# Autodesk Inventor assembly: wing_MIR
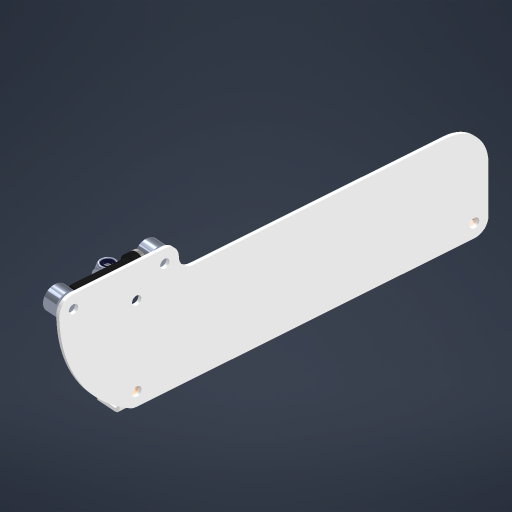
[picture p0: Inventor's stored thumbnail of the model, 512x512]
Saved by Autodesk Inventor 2024 (Build 280153000, 153)
## iProperties
Created: 2023-11-03
Part Number: wing_MIR
Document SubType Name: Assembly
Designer: avere
Author: avere
## Documents named in this file (11)
- C:\Users\avere\Documents\rbp_cad\zoomba_v0.1\chassis\wing_MIR.iam
- C:\Users\avere\Documents\rbp_cad\zoomba_v0.1\chassis\custom_parts\sled_MIR.ipt
- C:\Users\avere\Documents\rbp_cad\VEX-CAD-Inventor-1.41\Motion\Shaft LS\Shaft Collar ipts\Shaft Collar No Screw_MIR.ipt
- C:\Users\avere\Documents\rbp_cad\VEX-CAD-Inventor-1.41\Structure\Angle\Aluminum 1x1\Alu Angle 1x1x13_MIR.ipt
- C:\Users\avere\Documents\rbp_cad\VEX-CAD-Inventor-1.41\Structure\Standoff\Standoff 1.00.ipt
- C:\Users\avere\Documents\rbp_cad\VEX-CAD-Inventor-1.41\Structure\Standoff.ipt
- C:\Users\avere\Documents\rbp_cad\VEX-CAD-Inventor-1.41\Motion\Spacers\Spacer Nylon .375 OD\NSpacer .375 OD x .125.ipt
- C:\Users\avere\Documents\rbp_cad\VEX-CAD-Inventor-1.41\Motion\Spacers\Spacer Nylon .375 OD.ipt
- C:\Users\avere\Documents\rbp_cad\VEX-CAD-Inventor-1.41\Motion\Spacers\Washer Steel\SWasher .375 OD x .062500.ipt
- C:\Users\avere\Documents\rbp_cad\VEX-CAD-Inventor-1.41\Motion\Spacers\Washer Steel.ipt
- C:\Users\avere\Documents\rbp_cad\VEX-CAD-Inventor-1.41\Structure\Hardware\Nut Thin Nylock_MIR.ipt
## Components (10 placed, 7 different names)
1. sled_MIR:1 — Insert:10, Mate:4, Insert:11, Mate:5
2. Shaft Collar No Screw_MIR:1 — Insert:9, Insert:12
3. Shaft Collar No Screw_MIR:2 — Insert:9, Insert:8
4. Alu Angle 1x1x13_MIR:1 — Insert:10, Mate:4, Insert:12
5. Shaft Collar No Screw_MIR:3 — Mate:3, Insert:5, Insert:11
6. Shaft Collar No Screw_MIR:4 — Mate:3, Mate:5
7. Standoff 1.00:1 — Insert:5, Insert:4
8. NSpacer .375 OD x .125:1 — Insert:4, Insert:3
9. SWasher .375 OD x .062500:1 — Insert:3
10. Nut Thin Nylock_MIR:1 — Insert:8
## Relationships (11: Insert 8, Mate 3)
- Insert:9 (31.75 mm): Shaft Collar No Screw_MIR:1 ↔ Shaft Collar No Screw_MIR:2
- Mate:3: Shaft Collar No Screw_MIR:3 ↔ Shaft Collar No Screw_MIR:4
- Insert:5: Shaft Collar No Screw_MIR:3 ↔ Standoff 1.00:1
- Insert:4: Standoff 1.00:1 ↔ NSpacer .375 OD x .125:1
- Insert:3: NSpacer .375 OD x .125:1 ↔ SWasher .375 OD x .062500:1
- Insert:8: Shaft Collar No Screw_MIR:2 ↔ Nut Thin Nylock_MIR:1
- Insert:10: sled_MIR:1 ↔ Alu Angle 1x1x13_MIR:1
- Mate:4: sled_MIR:1 ↔ Alu Angle 1x1x13_MIR:1
- Insert:11 (1.5875 mm): sled_MIR:1 ↔ Shaft Collar No Screw_MIR:3
- Mate:5: sled_MIR:1 ↔ Shaft Collar No Screw_MIR:4
- Insert:12 (6.35 mm): Shaft Collar No Screw_MIR:1 ↔ Alu Angle 1x1x13_MIR:1
